# Autodesk Inventor assembly: T2601_EG
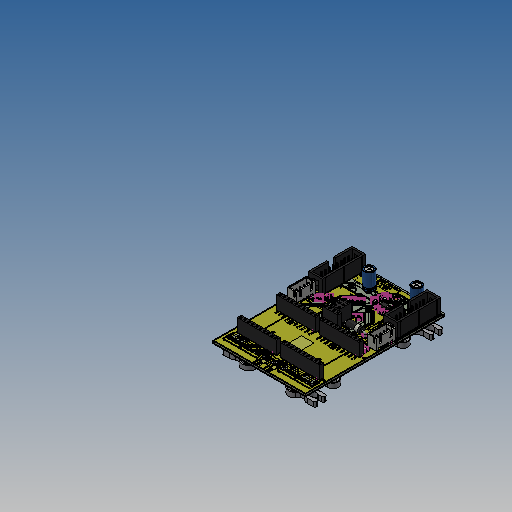
[picture p0: Inventor's stored thumbnail of the model, 512x512]
Saved by Autodesk Inventor 2025.3 (Build 293356000, 356)
## iProperties
Created: 2026-09-18
Part Number: T2601_EG
Project: Nom Projet
Description: Ens. Nom Ensemble
Document SubType Name: Assembly
Designer: jules
Mass: 0.019626 g
Surface Area: 471.188 cm^2
Volume: 19.626 cm^3
Density: 0.001 g/cm^3
Author: jules
## Documents named in this file (3)
- C:\Users\jules\OneDrive\PCB_Perso\T2601_APIArduino\T2601_Mecanique\T2601_EG.iam
- C:\Users\jules\OneDrive\PCB_Perso\T2601_APIArduino\T2601_Mecanique\T2601_ExtentionBoard\T2601_ExtentionBoard\T2601_ExtentionBoard.iam
- C:\Users\jules\OneDrive\PCB_Perso\T2601_APIArduino\T2601_Mecanique\T2601_BaseP30.ipt
## Components (2 placed, 2 different names)
1. T2601_ExtentionBoard:1 [sub-assembly] — Placage:1, Placage:2, Placage:3
2. T2601_BaseP30:1 — Placage:1, Placage:2, Placage:3
## Relationships (3: Mate 3)
- Placage:1 [Mate]: T2601_ExtentionBoard:1 ↔ T2601_BaseP30:1
- Placage:2 [Mate]: T2601_ExtentionBoard:1 ↔ T2601_BaseP30:1
- Placage:3 [Mate]: T2601_ExtentionBoard:1 ↔ T2601_BaseP30:1
